# Autodesk Inventor assembly: 大粗轴四方轴套反装套
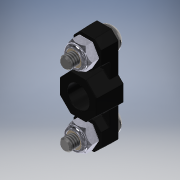
[picture p0: Inventor's stored thumbnail of the model, 180x180]
Saved by Autodesk Inventor 2019.4 (Build 234330000, 330)
## iProperties
Created: 2019-03-26
Part Number: 大粗轴四方轴套反装套
Material: 常规
Document SubType Name: Assembly
Designer: aresp
Mass: 10.3463 g
Surface Area: 29.8355 cm^2
Volume: 2.87965 cm^3
Density: 3.59289 g/cm^3
Author: aresp
## Documents named in this file (4)
- D:\towerTakeOverCad\ncrCadLib\大粗轴四方轴套反装套.iam
- D:\towerTakeOverCad\ncrCadLib\垫片轴套大白等\High Strength Shaft Bearing.ipt
- D:\towerTakeOverCad\ncrCadLib\螺丝螺帽\Nut 8-32 Nylock.ipt
- D:\towerTakeOverCad\ncrCadLib\螺丝螺帽\Screw 8-32 x 0.625'' - Black.ipt
## Components (5 placed, 3 different names)
1. High Strength Shaft Bearing:1
2. Nut 8-32 Nylock:1
3. Nut 8-32 Nylock:2
4. Screw 8-32 x 0.625'' - Black:1
5. Screw 8-32 x 0.625'' - Black:2
## Relationships (6: Mate 6)
- [Mate]: High Strength Shaft Bearing:1 ↔ Screw 8-32 x 0.625'' - Black:1
- [Mate]: High Strength Shaft Bearing:1 ↔ Screw 8-32 x 0.625'' - Black:2
- [Mate]: High Strength Shaft Bearing:1 ↔ Nut 8-32 Nylock:2
- [Mate]: High Strength Shaft Bearing:1 ↔ Nut 8-32 Nylock:1
- [Mate]: Nut 8-32 Nylock:2 ↔ Screw 8-32 x 0.625'' - Black:1
- [Mate]: Nut 8-32 Nylock:1 ↔ Screw 8-32 x 0.625'' - Black:2
